# Autodesk Inventor assembly: finalStagesAssembly
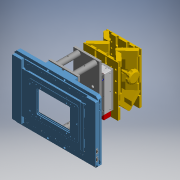
[picture p0: Inventor's stored thumbnail of the model, 180x180]
Saved by Autodesk Inventor 2016 (Build 200138000, 138)
## iProperties
Created: 2016-09-30
Part Number: finalStagesAssembly
Document SubType Name: Assembly
Designer: sims01
Author: sims01
## Documents named in this file (6)
- H:\Documents\LSFM_3\setup\mechanical\design\lsfm3_mechDesign\finalStagesAssembly.iam
- H:\Documents\LSFM_3\setup\mechanical\design\lsfm3_mechDesign\jackAssembly.iam
- H:\Documents\LSFM_3\setup\mechanical\design\lsfm3_mechDesign\zStagePostAttach.ipt
- H:\Documents\LSFM_3\setup\mechanical\design\lsfm3_mechDesign\stageMountingPost.ipt
- H:\Documents\LSFM_3\setup\mechanical\design\lsfm3_mechDesign\xyStagePostAttach.ipt
- H:\Documents\LSFM_3\setup\mechanical\design\lsfm3_mechDesign\piStage_XY.ipt
## Components (9 placed, 5 different names)
1. jackAssembly:1 [sub-assembly] — Rigid:1
2. zStagePostAttach:1 — Rigid:1, Rigid:2, Rigid:3, Rigid:4, Rigid:5
3. stageMountingPost:1 — Rigid:5, Rigid:6
4. stageMountingPost:2 — Rigid:4
5. stageMountingPost:3 — Rigid:2
6. stageMountingPost:4 — Rigid:3, Rotational:1
7. xyStagePostAttach:1 — Rigid:6, Rigid:7
8. xyStagePostAttach:2 — Rotational:1
9. piStage_XY:1 — Rigid:7
## Relationships (8: WeldJoint 7, RevoluteJoint 1)
- Rigid:1 [WeldJoint]: jackAssembly:1 ↔ zStagePostAttach:1
- Rigid:2 [WeldJoint]: zStagePostAttach:1 ↔ stageMountingPost:3
- Rigid:3 [WeldJoint]: zStagePostAttach:1 ↔ stageMountingPost:4
- Rigid:4 [WeldJoint]: zStagePostAttach:1 ↔ stageMountingPost:2
- Rigid:5 [WeldJoint]: zStagePostAttach:1 ↔ stageMountingPost:1
- Rigid:6 [WeldJoint]: stageMountingPost:1 ↔ xyStagePostAttach:1
- Rotational:1 [RevoluteJoint]: stageMountingPost:4 ↔ xyStagePostAttach:2
- Rigid:7 [WeldJoint]: xyStagePostAttach:1 ↔ piStage_XY:1
